# Autodesk Inventor assembly: Arm Differential Knuckle
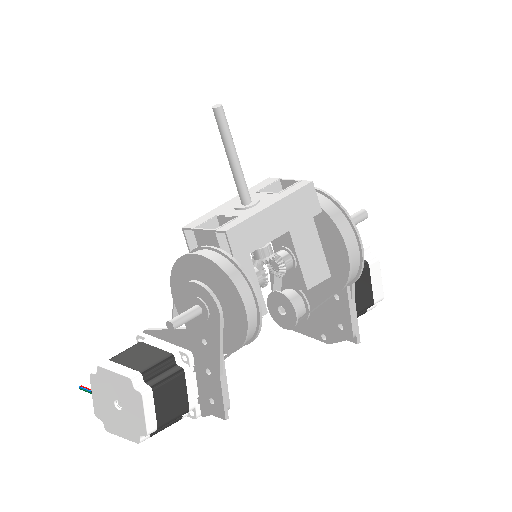
[picture p0: Inventor's stored thumbnail of the model, 512x512]
Saved by Autodesk Inventor 2025.2 (Build 292293000, 293)
## iProperties
Created: 2025-02-04
Part Number: Arm Differential Knuckle
Document SubType Name: Assembly
Designer: Jakeg
Author: Jakeg
## Documents named in this file (13)
- C:\Users\Jakeg\OneDrive\Documents\GitHub\BehrendURCMechanical\CAD\Arm\Knuckle\Arm Differential Knuckle.iam
- C:\Users\Jakeg\OneDrive\Documents\GitHub\BehrendURCMechanical\CAD\Arm\ARM MAIN\Arm Plates\Arm Plate.ipt
- C:\Users\Jakeg\OneDrive\Documents\GitHub\BehrendURCMechanical\CAD\Arm\Knuckle\2600N1_Metal Miter Gear.ipt
- C:\Users\Jakeg\OneDrive\Documents\GitHub\BehrendURCMechanical\CAD\Arm\Knuckle\23HE22-2804S.ipt
- C:\Users\Jakeg\OneDrive\Documents\GitHub\BehrendURCMechanical\CAD\Arm\Knuckle\Diff 8mm Bearing.ipt
- C:\Users\Jakeg\OneDrive\Documents\GitHub\BehrendURCMechanical\CAD\Arm\Knuckle\Diff Side Bar.ipt
- C:\Users\Jakeg\OneDrive\Documents\GitHub\BehrendURCMechanical\CAD\Arm\Knuckle\Diff Top Bar.ipt
- C:\Users\Jakeg\OneDrive\Documents\GitHub\BehrendURCMechanical\CAD\Arm\Knuckle\Diff Side Shafts.ipt
- C:\Users\Jakeg\OneDrive\Documents\GitHub\BehrendURCMechanical\CAD\Arm\Knuckle\Diff Output Shaft.ipt
- C:\Users\Jakeg\OneDrive\Documents\GitHub\BehrendURCMechanical\CAD\Arm\Knuckle\Diff Large Pulley.ipt
- C:\Users\Jakeg\OneDrive\Documents\GitHub\BehrendURCMechanical\CAD\Arm\Knuckle\Diff Small Pulley.ipt
- C:\Users\Jakeg\OneDrive\Documents\GitHub\BehrendURCMechanical\CAD\Arm\Knuckle\Diff Motor Belts.ipt
- C:\Users\Jakeg\OneDrive\Documents\GitHub\BehrendURCMechanical\CAD\Arm\Knuckle\Diff Motor Bracket.ipt
## Components (29 placed, 12 different names)
1. arm plate:1 — Mate:1, Mate:2, Mate:29, Mate:47, Mate:49, Mate:50
2. arm plate:2 — Mate:3, Mate:4, Mate:29, Mate:53, Mate:54, Mate:55
3. 2600N1_Metal Miter Gear:1 — Mate:15, Flush:6, Rigid:1
4. 2600N1_Metal Miter Gear:2 — Flush:2, Flush:5, Rigid:3
5. 2600N1_Metal Miter Gear:3 — Flush:7, Mate:60, Rigid:2
6. 23HE22-2804S:1 — Mate:32, Mate:56, Rigid:4
7. 23HE22-2804S:2 — Mate:33, Mate:51, Rigid:5
8. Diff 8mm Bearing:1 — Mate:1, Mate:2, Mate:6, Mate:7, Mate:16, Mate:27
9. Diff 8mm Bearing:2 — Mate:3, Mate:4, Mate:5, Mate:7, Mate:17, Mate:28
10. Diff Side Bar:1 — Mate:5, Mate:10, Mate:11, Mate:22, Flush:3, Mate:30, Flush:9
11. Diff Side Bar:2 — Mate:6, Mate:12, Mate:13, Mate:20, Flush:4, Mate:31, Flush:8
12. Diff Top Bar:1 — Mate:10, Mate:11, Mate:12, Mate:13, Flush:1, Mate:40, Mate:42, Flush:8, Rotational:3
13. Diff Side Shafts:1 — Mate:17, Mate:21, Mate:23, Mate:25, Flush:6, Rigid:1
14. Diff Side Shafts:2 — Mate:16, Mate:19, Mate:24, Mate:26, Flush:5, Rigid:3
15. Diff Output Shaft:1 — Flush:7, Mate:39, Mate:41, Rigid:2
16. Diff 8mm Bearing:3 — Mate:23, Flush:3
17. Diff 8mm Bearing:4 — Mate:24, Flush:4
18. Diff 8mm Bearing:5 — Mate:19, Mate:20
19. Diff 8mm Bearing:6 — Mate:21, Mate:22
20. Diff Large Pulley:1 — Mate:25, Mate:28, Mate:30, Mate:34, Mate:37
21. Diff Large Pulley:2 — Mate:26, Mate:27, Mate:31, Mate:35, Mate:43
22. Diff Small Pulley:1 — Mate:32, Mate:36
23. Diff Small Pulley:2 — Mate:33, Mate:38
24. Diff Motor Belts:1 — Mate:34, Mate:36, Mate:37
25. Diff Motor Belts:2 — Mate:35, Mate:38, Mate:43
26. Diff 8mm Bearing:7 — Mate:39, Mate:40, Rotational:3
27. Diff 8mm Bearing:8 — Mate:41, Mate:42
28. Diff Motor Bracket:1 — Mate:53, Mate:54, Mate:55, Mate:56, Rigid:4
29. Diff Motor Bracket:2 — Mate:47, Mate:49, Mate:50, Mate:51, Rigid:5
## Relationships (63: Mate 48, Flush 9, WeldJoint 5, RevoluteJoint 1)
- Mate:1: arm plate:1 ↔ Diff 8mm Bearing:1
- Mate:2: arm plate:1 ↔ Diff 8mm Bearing:1
- Mate:3: arm plate:2 ↔ Diff 8mm Bearing:2
- Mate:4: arm plate:2 ↔ Diff 8mm Bearing:2
- Mate:5: Diff 8mm Bearing:2 ↔ Diff Side Bar:1
- Mate:6: Diff 8mm Bearing:1 ↔ Diff Side Bar:2
- Mate:7: Diff 8mm Bearing:1 ↔ Diff 8mm Bearing:2
- Mate:10: Diff Side Bar:1 ↔ Diff Top Bar:1
- Mate:11: Diff Side Bar:1 ↔ Diff Top Bar:1
- Mate:12: Diff Side Bar:2 ↔ Diff Top Bar:1
- Mate:13: Diff Side Bar:2 ↔ Diff Top Bar:1
- Flush:1 (-46.228 mm): Diff Top Bar:1
- Flush:2 (20 mm): 2600N1_Metal Miter Gear:2
- Mate:15 (-20 mm): 2600N1_Metal Miter Gear:1
- Mate:16: Diff 8mm Bearing:1 ↔ Diff Side Shafts:2
- Mate:17: Diff 8mm Bearing:2 ↔ Diff Side Shafts:1
- Mate:19: Diff Side Shafts:2 ↔ Diff 8mm Bearing:5
- Mate:20: Diff Side Bar:2 ↔ Diff 8mm Bearing:5
- Mate:21: Diff Side Shafts:1 ↔ Diff 8mm Bearing:6
- Mate:22: Diff Side Bar:1 ↔ Diff 8mm Bearing:6
- Mate:23: Diff Side Shafts:1 ↔ Diff 8mm Bearing:3
- Flush:3: Diff Side Bar:1 ↔ Diff 8mm Bearing:3
- Mate:24: Diff Side Shafts:2 ↔ Diff 8mm Bearing:4
- Flush:4: Diff Side Bar:2 ↔ Diff 8mm Bearing:4
- Mate:25: Diff Side Shafts:1 ↔ Diff Large Pulley:1
- Mate:26: Diff Side Shafts:2 ↔ Diff Large Pulley:2
- Mate:27: Diff 8mm Bearing:1 ↔ Diff Large Pulley:2
- Mate:28: Diff 8mm Bearing:2 ↔ Diff Large Pulley:1
- Mate:29: arm plate:1 ↔ arm plate:2
- Mate:30: Diff Side Bar:1 ↔ Diff Large Pulley:1
- Mate:31: Diff Side Bar:2 ↔ Diff Large Pulley:2
- Flush:5: 2600N1_Metal Miter Gear:2 ↔ Diff Side Shafts:2
- Flush:6: 2600N1_Metal Miter Gear:1 ↔ Diff Side Shafts:1
- Flush:7: 2600N1_Metal Miter Gear:3 ↔ Diff Output Shaft:1
- Mate:32: 23HE22-2804S:1 ↔ Diff Small Pulley:1
- Mate:33: 23HE22-2804S:2 ↔ Diff Small Pulley:2
- Mate:34: Diff Large Pulley:1 ↔ Diff Motor Belts:1
- Mate:35: Diff Large Pulley:2 ↔ Diff Motor Belts:2
- Mate:36: Diff Small Pulley:1 ↔ Diff Motor Belts:1
- Mate:37 (1.0795 mm): Diff Large Pulley:1 ↔ Diff Motor Belts:1
- Mate:38: Diff Small Pulley:2 ↔ Diff Motor Belts:2
- Mate:39: Diff Output Shaft:1 ↔ Diff 8mm Bearing:7
- Mate:40: Diff Top Bar:1 ↔ Diff 8mm Bearing:7
- Mate:41: Diff Output Shaft:1 ↔ Diff 8mm Bearing:8
- Mate:42: Diff Top Bar:1 ↔ Diff 8mm Bearing:8
- Mate:43 (1.0795 mm): Diff Large Pulley:2 ↔ Diff Motor Belts:2
- Mate:47: arm plate:1 ↔ Diff Motor Bracket:2
- Mate:49: arm plate:1 ↔ Diff Motor Bracket:2
- Mate:50: arm plate:1 ↔ Diff Motor Bracket:2
- Mate:51: 23HE22-2804S:2 ↔ Diff Motor Bracket:2
- Mate:53: arm plate:2 ↔ Diff Motor Bracket:1
- Mate:54: arm plate:2 ↔ Diff Motor Bracket:1
- Mate:55: arm plate:2 ↔ Diff Motor Bracket:1
- Mate:56: 23HE22-2804S:1 ↔ Diff Motor Bracket:1
- Flush:8: Diff Side Bar:2 ↔ Diff Top Bar:1
- Flush:9 (-25.4 mm): Diff Side Bar:1
- Mate:60 (-19.9898 mm): 2600N1_Metal Miter Gear:3
- Rotational:3 [RevoluteJoint]: Diff Top Bar:1 ↔ Diff 8mm Bearing:7
- Rigid:1 [WeldJoint]: 2600N1_Metal Miter Gear:1 ↔ Diff Side Shafts:1
- Rigid:2 [WeldJoint]: 2600N1_Metal Miter Gear:3 ↔ Diff Output Shaft:1
- Rigid:3 [WeldJoint]: 2600N1_Metal Miter Gear:2 ↔ Diff Side Shafts:2
- Rigid:4 [WeldJoint]: 23HE22-2804S:1 ↔ Diff Motor Bracket:1
- Rigid:5 [WeldJoint]: 23HE22-2804S:2 ↔ Diff Motor Bracket:2
